# Autodesk Inventor assembly: CableChain_Clamp
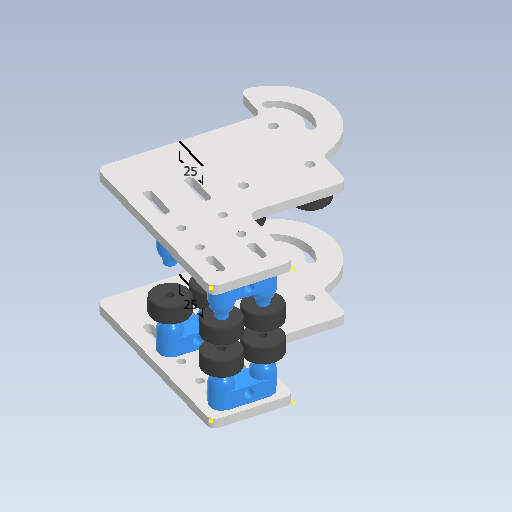
[picture p0: Inventor's stored thumbnail of the model, 512x512]
Saved by Autodesk Inventor 2021 (Build 250183000, 183)
## iProperties
Created: 2021-12-21
Part Number: CableChain_Clamp
Document SubType Name: Assembly
Designer: Jorian Brusind
Author: Jorian Brusind
## Documents named in this file (5)
- C:\Users\Jorian Brusind\Documents\GitHub\PersonalProjects\HyperRail\Inventor Files\CableChain_Clamp.iam
- C:\Users\Jorian Brusind\Documents\GitHub\PersonalProjects\HyperRail\Inventor Files\CableChain_Plate.ipt
- C:\Users\Jorian Brusind\Documents\GitHub\PersonalProjects\HyperRail\Inventor Files\11mm_BearingWheel.ipt
- C:\Users\Jorian Brusind\Documents\GitHub\PersonalProjects\HyperRail\Inventor Files\4mm_Roller_Spacer_simple.ipt
- C:\Users\Jorian Brusind\Documents\GitHub\PersonalProjects\HyperRail\Inventor Files\5mm_Spacer.ipt
## Components (18 placed, 4 different names)
1. CableChain_Plate:1 — Mate:23, Mate:24, Mate:25, Mate:28, Mate:32, Mate:33, Mate:34, Mate:35, Flush:3
2. CableChain_Plate:2 — Mate:3, Mate:5, Mate:19, Mate:20, Mate:21, Mate:22, Flush:3
3. 11mm_BearingWheel:1 — Mate:6, Mate:26
4. 4mm_Roller_Spacer_simple:1 — Mate:2, Mate:3, Mate:4, Mate:5, Mate:6, Mate:22
5. 11mm_BearingWheel:2 — Mate:2, Mate:4, Mate:27, Mate:31
6. 11mm_BearingWheel:3 — Mate:19, Mate:29
7. 4mm_Roller_Spacer_simple:2 — Mate:20, Mate:21
8. 11mm_BearingWheel:4 — Mate:30
9. 11mm_BearingWheel:5 — Mate:27, Mate:31
10. 4mm_Roller_Spacer_simple:3 — Mate:23, Mate:24, Mate:25
11. 11mm_BearingWheel:6 — Mate:26
12. 4mm_Roller_Spacer_simple:4 — Mate:28, Mate:29, Mate:30
13. 5mm_Spacer:1 — Mate:33, Flush:2, Mate:37, Mate:41
14. 5mm_Spacer:2 — Mate:34, Flush:1, Mate:38, Mate:39
15. 5mm_Spacer:3 — Mate:32, Flush:1, Flush:2, Mate:35, Mate:36, Mate:40
16. 11mm_BearingWheel:7 — Mate:36, Mate:40
17. 11mm_BearingWheel:8 — Mate:37, Mate:41
18. 11mm_BearingWheel:9 — Mate:38, Mate:39
## Relationships (40: Mate 37, Flush 3)
- [Mate]: 11mm_BearingWheel:1 ↔ 4mm_Roller_Spacer_simple:1
- Mate:2: 4mm_Roller_Spacer_simple:1 ↔ 11mm_BearingWheel:2
- Mate:3 (2.5 mm): CableChain_Plate:2 ↔ 4mm_Roller_Spacer_simple:1
- Mate:4: 4mm_Roller_Spacer_simple:1 ↔ 11mm_BearingWheel:2
- Mate:5: CableChain_Plate:2 ↔ 4mm_Roller_Spacer_simple:1
- Mate:6: 11mm_BearingWheel:1 ↔ 4mm_Roller_Spacer_simple:1
- [Mate]: 11mm_BearingWheel:3 ↔ 4mm_Roller_Spacer_simple:2
- [Mate]: 4mm_Roller_Spacer_simple:2 ↔ 11mm_BearingWheel:4
- [Mate]: 4mm_Roller_Spacer_simple:2 ↔ 11mm_BearingWheel:4
- [Mate]: 11mm_BearingWheel:3 ↔ 4mm_Roller_Spacer_simple:2
- [Mate]: 11mm_BearingWheel:5 ↔ 4mm_Roller_Spacer_simple:3
- [Mate]: 4mm_Roller_Spacer_simple:3 ↔ 11mm_BearingWheel:6
- [Mate]: 4mm_Roller_Spacer_simple:3 ↔ 11mm_BearingWheel:6
- [Mate]: 11mm_BearingWheel:5 ↔ 4mm_Roller_Spacer_simple:3
- Mate:19 (2.5 mm): CableChain_Plate:2 ↔ 11mm_BearingWheel:3
- Mate:20: CableChain_Plate:2 ↔ 4mm_Roller_Spacer_simple:2
- Mate:21 (2.5 mm): CableChain_Plate:2 ↔ 4mm_Roller_Spacer_simple:2
- Mate:22 (2.5 mm): CableChain_Plate:2 ↔ 4mm_Roller_Spacer_simple:1
- Mate:23: CableChain_Plate:1 ↔ 4mm_Roller_Spacer_simple:3
- Mate:24 (2.5 mm): CableChain_Plate:1 ↔ 4mm_Roller_Spacer_simple:3
- Mate:25 (2.5 mm): CableChain_Plate:1 ↔ 4mm_Roller_Spacer_simple:3
- Mate:26: 11mm_BearingWheel:1 ↔ 11mm_BearingWheel:6
- Mate:27: 11mm_BearingWheel:2 ↔ 11mm_BearingWheel:5
- Mate:28: CableChain_Plate:1 ↔ 4mm_Roller_Spacer_simple:4
- Mate:29: 11mm_BearingWheel:3 ↔ 4mm_Roller_Spacer_simple:4
- Mate:30: 11mm_BearingWheel:4 ↔ 4mm_Roller_Spacer_simple:4
- Mate:31 (10 mm): 11mm_BearingWheel:2 ↔ 11mm_BearingWheel:5
- Mate:32: CableChain_Plate:1 ↔ 5mm_Spacer:3
- Mate:33: CableChain_Plate:1 ↔ 5mm_Spacer:1
- Mate:34: CableChain_Plate:1 ↔ 5mm_Spacer:2
- Flush:1: 5mm_Spacer:2 ↔ 5mm_Spacer:3
- Flush:2: 5mm_Spacer:1 ↔ 5mm_Spacer:3
- Mate:35: CableChain_Plate:1 ↔ 5mm_Spacer:3
- Mate:36: 5mm_Spacer:3 ↔ 11mm_BearingWheel:7
- Mate:37: 5mm_Spacer:1 ↔ 11mm_BearingWheel:8
- Mate:38: 5mm_Spacer:2 ↔ 11mm_BearingWheel:9
- Mate:39: 5mm_Spacer:2 ↔ 11mm_BearingWheel:9
- Mate:40: 5mm_Spacer:3 ↔ 11mm_BearingWheel:7
- Mate:41: 5mm_Spacer:1 ↔ 11mm_BearingWheel:8
- Flush:3: CableChain_Plate:1 ↔ CableChain_Plate:2
## Named parameters: d15_d95 = 0 mm, d16_d10 = 0 mm, d17_d12 = 0 mm, d18_d14 = 0 mm, d19_d95 = 0 mm, d20_d10 = 0 mm, d21_d12 = 0 mm, d22_d14 = 0 mm
